# Autodesk Inventor assembly: Module Assembly
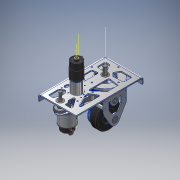
[picture p0: Inventor's stored thumbnail of the model, 180x180]
Saved by Autodesk Inventor 2019.4 (Build 234330000, 330)
## iProperties
Created: 2019-11-29
Part Number: Module Assembly
Document SubType Name: Assembly
Designer: admin
Mass: 4044.05 g
Surface Area: 4877.01 cm^2
Volume: 1359.37 cm^3
Density: 2.97495 g/cm^3
Author: admin
## Documents named in this file (30)
- C:\Users\admin\Desktop\FRC 2020 Engineering\GitHub\7738-CAD-prep\Swerve Module\Module Assembly.iam
- C:\Users\admin\Desktop\FRC 2020 Engineering\GitHub\7738-CAD-prep\Swerve Module\100mm Traction Wheel StandIn.ipt
- C:\Users\admin\Desktop\FRC 2020 Engineering\GitHub\7738-CAD-prep\Swerve Module\Falcon_500_Powered_by_Talon_FX_217-6515.iam
- C:\Users\admin\Desktop\FRC 2020 Engineering\GitHub\7738-CAD-prep\Swerve Module\U Bend.ipt
- C:\Users\admin\Desktop\FRC 2020 Engineering\GitHub\7738-CAD-prep\Swerve Module\Bearing.ipt
- C:\Users\admin\Desktop\FRC 2020 Engineering\GitHub\7738-CAD-prep\Swerve Module\Module Assembly\Design Accelerator\Synchronous Belts Transmission3.iam
- C:\Users\admin\Desktop\FRC 2020 Engineering\GitHub\7738-CAD-prep\Swerve Module\Module Assembly\Design Accelerator\Synchronous Belts Transmission4.iam
- C:\Users\admin\Desktop\FRC 2020 Engineering\GitHub\7738-CAD-prep\Swerve Module\Top Plate.ipt
- C:\Users\admin\Desktop\FRC 2020 Engineering\GitHub\7738-CAD-prep\Swerve Module\F6802.ipt
- C:\Users\admin\Desktop\FRC 2020 Engineering\GitHub\7738-CAD-prep\Swerve Module\Main Vert Axle.ipt
- C:\Users\admin\Desktop\FRC 2020 Engineering\GitHub\7738-CAD-prep\Swerve Module\Module Assembly\Design Accelerator\Bevel Gears2.iam
- C:\Users\admin\Desktop\FRC 2020 Engineering\GitHub\7738-CAD-prep\Swerve Module\Module Assembly\Design Accelerator\Spur Gears4.iam
- C:\Users\admin\Desktop\FRC 2020 Engineering\GitHub\7738-CAD-prep\Swerve Module\30t_Aluminum_Spur_Gear_20_DP_1_2_Hex_Bore_217-2705.ipt
- C:\Users\admin\Desktop\FRC 2020 Engineering\GitHub\7738-CAD-prep\Swerve Module\14T_Steel_Spur_Gear_20_DP_Falcon_Motor_217-6922.ipt
- C:\Users\admin\Desktop\FRC 2020 Engineering\GitHub\7738-CAD-prep\Swerve Module\EB38S6 Encoder.ipt
- C:\Users\admin\Desktop\FRC 2020 Engineering\GitHub\7738-CAD-prep\Swerve Module\F6800Z 10mm ID Flange.ipt
- C:\Users\admin\Desktop\FRC 2020 Engineering\GitHub\7738-CAD-prep\Swerve Module\Bevel - Spur Axle.ipt
- C:\Users\admin\Desktop\FRC 2020 Engineering\GitHub\7738-CAD-prep\Swerve Module\Wheel - Spur Axle.ipt
- C:\Users\admin\Desktop\FRC 2020 Engineering\GitHub\7738-CAD-prep\Swerve Module\27-1 Gearbox.ipt
- C:\Users\admin\Desktop\FRC 2020 Engineering\GitHub\7738-CAD-prep\Swerve Module\775pro_217-4347.ipt
- C:\Users\admin\Desktop\FRC 2020 Engineering\GitHub\7738-CAD-prep\Swerve Module\Gear - Drive Axle.ipt
- C:\Users\admin\Desktop\FRC 2020 Engineering\GitHub\7738-CAD-prep\775 Mounting plate.ipt
- C:\Users\admin\Desktop\FRC 2020 Engineering\GitHub\7738-CAD-prep\Swerve Module\Motor Mount Plate.ipt
- C:\Users\admin\Desktop\FRC 2020 Engineering\GitHub\7738-CAD-prep\Swerve Module\Spacer.ipt
- C:\Users\admin\Desktop\FRC 2020 Engineering\GitHub\7738-CAD-prep\Swerve Module\Spacer 2.ipt
- C:\Users\admin\Desktop\FRC 2020 Engineering\GitHub\7738-CAD-prep\Swerve Module\Module Assembly\Design Accelerator\Key Connection1.iam
- C:\Users\admin\Desktop\FRC 2020 Engineering\GitHub\7738-CAD-prep\Swerve Module\Module Assembly\Design Accelerator\Key Connection3.iam
- C:\Users\admin\Desktop\FRC 2020 Engineering\GitHub\7738-CAD-prep\Swerve Module\Module Assembly\Design Accelerator\Key Connection2.iam
- C:\Users\admin\Desktop\FRC 2020 Engineering\GitHub\7738-CAD-prep\Swerve Module\Module Assembly\Design Accelerator\Key Connection5.iam
- C:\Users\admin\Desktop\FRC 2020 Engineering\GitHub\7738-CAD-prep\Swerve Module\Module Assembly\Design Accelerator\Key Connection7.iam
## Components (43 placed, 24 different names)
1. 100mm Traction Wheel StandIn:1 — Mate:82, Mate:86
2. Falcon_500_Powered_by_Talon_FX_217-6515:1 [sub-assembly] — Mate:12, Mate:13, Mate:21, Mate:33, Flush:3, Mate:34, Mate:35
3. Synchronous Belts Transmission:1 [sub-assembly] — Mate:1, Mate:6, Mate:20, Mate:25, Mate:28, Mate:29, Mate:72, Mate:73, Mate:91
4. Synchronous Belts Transmission:2 [sub-assembly] — Mate:14, Mate:22, Angle:1, Angle:2
5. F6802:2 — Mate:80, Mate:81
6. F6802:3 — Mate:71, Mate:74, Mate:75
7. Main Vert Axle:1 — Mate:3, Flush:1, Angle:2, Mate:71
8. Bevel Gears:2 [sub-assembly] — Mate:2, Mate:3, Flush:1, Mate:57, Angle:3, Angle:4
9. Spur Gears:3 [sub-assembly] — Mate:86, Flush:4, Angle:5, Mate:92
10. 30t_Aluminum_Spur_Gear_20_DP_1_2_Hex_Bore_217-2705:1 — Mate:11, Mate:13, Flush:2, Mate:18
11. 14T_Steel_Spur_Gear_20_DP_Falcon_Motor_217-6922:1 — Mate:12, Flush:2
12. F6800Z 10mm ID Flange:1 — Mate:58, Mate:63
13. F6800Z 10mm ID Flange:2 — Mate:59, Mate:62, Mate:76, Mate:77
14. Bevel - Spur Axle:2 — Mate:57, Mate:58, Mate:59, Mate:62, Mate:63, Flush:4, Angle:4, Angle:5, Mate:92
15. F6802:5 — Mate:67, Mate:70, Mate:78, Mate:79
16. Wheel - Spur Axle:1 — Mate:67, Mate:70, Mate:82
17. 27-1 Gearbox:1 — Mate:8, Mate:9, Mate:28, Mate:29, Mate:30, Mate:31
18. 775pro_217-4347:1 — Mate:8, Mate:9
19. EB38S6 Encoder:2 — Mate:6, Flush:3
20. F6802:6 — Mate:16
21. F6800Z 10mm ID Flange:3 — Mate:15, Mate:17, Mate:18, Mate:33
22. Gear - Drive Axle:1 — Mate:11, Mate:14, Mate:15, Mate:16, Mate:17, Mate:22, Angle:1
23. Bearing:1 — Mate:1, Mate:2, Mate:20, Mate:24
24. Top Plate:2 — Mate:24, Mate:25, Mate:83, Mate:84
25. 775 Mounting plate:1 — Mate:30, Mate:31
26. Motor Mount Plate:1 — Mate:34, Mate:35, Mate:37, Mate:38, Mate:39, Mate:40, Mate:53, Mate:54, Mate:55, Mate:56
27. Spacer:1 — Mate:37
28. Spacer:2 — Mate:38
29. Spacer:3 — Mate:40
30. Spacer:5 — Mate:39
31. Spacer 2:1 — Mate:87, Mate:90
32. Spacer 2:2 — Mate:88, Mate:89
33. Spacer 2:3 — Mate:94, Mate:96
34. Spacer 2:4 — Mate:93, Mate:95
35. Key Connection:1 [sub-assembly]
36. Spacer:6 — Mate:53, Mate:54
37. Spacer:7 — Mate:55, Mate:56
38. Key Connection:2 [sub-assembly] — Angle:3
39. U Bend:1 — Mate:72, Mate:73, Mate:74, Mate:75, Mate:76, Mate:77, Mate:78, Mate:79, Mate:80, Mate:81, Mate:87, Mate:88, Mate:89, Mate:90, Mate:91, Mate:93, Mate:94, Mate:95, Mate:96
40. F6802:7 — Mate:83, Mate:84
41. Key Connection:3 [sub-assembly]
42. Key Connection:4 [sub-assembly]
43. Key Connection:5 [sub-assembly]
## Relationships (75: Mate 66, Angle 5, Flush 4)
- Mate:1 (1 mm): Synchronous Belts Transmission:1 ↔ Bearing:1
- Mate:2: Bevel Gears:2 ↔ Bearing:1
- Mate:3: Main Vert Axle:1 ↔ Bevel Gears:2
- Flush:1 (-0.1 mm): Main Vert Axle:1 ↔ Bevel Gears:2
- Mate:6: Synchronous Belts Transmission:1 ↔ EB38S6 Encoder:2
- Mate:8: 27-1 Gearbox:1 ↔ 775pro_217-4347:1
- Mate:9: 27-1 Gearbox:1 ↔ 775pro_217-4347:1
- Mate:11: 30t_Aluminum_Spur_Gear_20_DP_1_2_Hex_Bore_217-2705:1 ↔ Gear - Drive Axle:1
- Mate:12: Falcon_500_Powered_by_Talon_FX_217-6515:1 ↔ 14T_Steel_Spur_Gear_20_DP_Falcon_Motor_217-6922:1
- Mate:13 (27.94 mm): Falcon_500_Powered_by_Talon_FX_217-6515:1 ↔ 30t_Aluminum_Spur_Gear_20_DP_1_2_Hex_Bore_217-2705:1
- Flush:2 (1 mm): 30t_Aluminum_Spur_Gear_20_DP_1_2_Hex_Bore_217-2705:1 ↔ 14T_Steel_Spur_Gear_20_DP_Falcon_Motor_217-6922:1
- Mate:14: Synchronous Belts Transmission:2 ↔ Gear - Drive Axle:1
- Mate:15: F6800Z 10mm ID Flange:3 ↔ Gear - Drive Axle:1
- Mate:16: F6802:6 ↔ Gear - Drive Axle:1
- Mate:17 (0.2 mm): F6800Z 10mm ID Flange:3 ↔ Gear - Drive Axle:1
- Mate:18 (0.2 mm): 30t_Aluminum_Spur_Gear_20_DP_1_2_Hex_Bore_217-2705:1 ↔ F6800Z 10mm ID Flange:3
- Mate:20: Synchronous Belts Transmission:1 ↔ Bearing:1
- Mate:21: Falcon_500_Powered_by_Talon_FX_217-6515:1
- Mate:22 (0.2 mm): Synchronous Belts Transmission:2 ↔ Gear - Drive Axle:1
- Mate:24 (1 mm): Bearing:1 ↔ Top Plate:2
- Mate:25: Synchronous Belts Transmission:1 ↔ Top Plate:2
- Mate:28: Synchronous Belts Transmission:1 ↔ 27-1 Gearbox:1
- Mate:29 (5.5 mm): Synchronous Belts Transmission:1 ↔ 27-1 Gearbox:1
- Mate:30: 27-1 Gearbox:1 ↔ 775 Mounting plate:1
- Mate:31: 27-1 Gearbox:1 ↔ 775 Mounting plate:1
- Mate:33 (5.2 mm): Falcon_500_Powered_by_Talon_FX_217-6515:1 ↔ F6800Z 10mm ID Flange:3
- Flush:3 (1 mm): Falcon_500_Powered_by_Talon_FX_217-6515:1 ↔ EB38S6 Encoder:2
- Mate:34: Falcon_500_Powered_by_Talon_FX_217-6515:1 ↔ Motor Mount Plate:1
- Mate:35: Falcon_500_Powered_by_Talon_FX_217-6515:1 ↔ Motor Mount Plate:1
- Mate:37: Motor Mount Plate:1 ↔ Spacer:1
- Mate:38: Motor Mount Plate:1 ↔ Spacer:2
- Mate:39: Motor Mount Plate:1 ↔ Spacer:5
- Mate:40: Motor Mount Plate:1 ↔ Spacer:3
- Angle:1 (84.5005 deg): Synchronous Belts Transmission:2 ↔ Gear - Drive Axle:1
- Mate:53: Motor Mount Plate:1 ↔ Spacer:6
- Mate:54 (0.2 mm): Motor Mount Plate:1 ↔ Spacer:6
- Mate:55: Motor Mount Plate:1 ↔ Spacer:7
- Mate:56 (0.2 mm): Motor Mount Plate:1 ↔ Spacer:7
- Angle:2 (111.4709 deg): Synchronous Belts Transmission:2 ↔ Main Vert Axle:1
- Mate:57: Bevel Gears:2 ↔ Bevel - Spur Axle:2
- Mate:58: F6800Z 10mm ID Flange:1 ↔ Bevel - Spur Axle:2
- Mate:59: F6800Z 10mm ID Flange:2 ↔ Bevel - Spur Axle:2
- Mate:62 (0.1 mm): F6800Z 10mm ID Flange:2 ↔ Bevel - Spur Axle:2
- Mate:63 (0.1 mm): F6800Z 10mm ID Flange:1 ↔ Bevel - Spur Axle:2
- Mate:67: F6802:5 ↔ Wheel - Spur Axle:1
- Mate:70 (0.2 mm): F6802:5 ↔ Wheel - Spur Axle:1
- Mate:71: F6802:3 ↔ Main Vert Axle:1
- Mate:72: Synchronous Belts Transmission:1 ↔ U Bend:1
- Mate:73: Synchronous Belts Transmission:1 ↔ U Bend:1
- Mate:74: F6802:3 ↔ U Bend:1
- Mate:75 (0.2 mm): F6802:3 ↔ U Bend:1
- Mate:76: F6800Z 10mm ID Flange:2 ↔ U Bend:1
- Mate:77 (0.2 mm): F6800Z 10mm ID Flange:2 ↔ U Bend:1
- Mate:78: F6802:5 ↔ U Bend:1
- Mate:79 (0.2 mm): F6802:5 ↔ U Bend:1
- Mate:80 (0.2 mm): F6802:2 ↔ U Bend:1
- Mate:81: F6802:2 ↔ U Bend:1
- Mate:82: 100mm Traction Wheel StandIn:1 ↔ Wheel - Spur Axle:1
- Mate:83: Top Plate:2 ↔ F6802:7
- Mate:84 (0.2 mm): Top Plate:2 ↔ F6802:7
- Mate:86 (4.7 mm): 100mm Traction Wheel StandIn:1 ↔ Spur Gears:3
- Flush:4 (-0.1 mm): Spur Gears:3 ↔ Bevel - Spur Axle:2
- Mate:87: Spacer 2:1 ↔ U Bend:1
- Mate:88: Spacer 2:2 ↔ U Bend:1
- Mate:89 (0.2 mm): Spacer 2:2 ↔ U Bend:1
- Mate:90 (0.2 mm): Spacer 2:1 ↔ U Bend:1
- Mate:91: Synchronous Belts Transmission:1 ↔ U Bend:1
- Angle:3 (89.8477 deg): Bevel Gears:2 ↔ Key Connection:2
- Angle:4 (49.7402 deg): Bevel Gears:2 ↔ Bevel - Spur Axle:2
- Angle:5 (132.0596 deg): Spur Gears:3 ↔ Bevel - Spur Axle:2
- Mate:92: Spur Gears:3 ↔ Bevel - Spur Axle:2
- Mate:93: Spacer 2:4 ↔ U Bend:1
- Mate:94: Spacer 2:3 ↔ U Bend:1
- Mate:95 (0.2 mm): Spacer 2:4 ↔ U Bend:1
- Mate:96 (0.2 mm): Spacer 2:3 ↔ U Bend:1
